# Autodesk Inventor assembly: Funnel Assembly
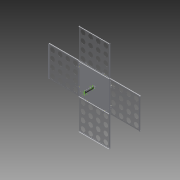
[picture p0: Inventor's stored thumbnail of the model, 180x180]
Saved by Autodesk Inventor 2014 (Build 180170000, 170)
## iProperties
Created: 2014-01-05
Part Number: Funnel Assembly
Document SubType Name: Assembly
Designer: Michael
Mass: 3587.59 g
Surface Area: 25589.4 cm^2
Volume: 1918.45 cm^3
Density: 1.87005 g/cm^3
Author: Michael
## Documents named in this file (5)
- C:\Users\Michael\Documents\Robotics\2014 Season\Funnel Catcher\Funnel Assembly.iam
- C:\Users\Michael\Documents\Robotics\2014 Season\Funnel Catcher\Funnel Plate Assembly.iam
- C:\Users\Michael\Documents\Robotics\2014 Season\Funnel Catcher\Flange for 3-4 in Piston.ipt
- C:\Users\Michael\Documents\Robotics\2014 Season\Funnel Catcher\9-16 in Pneumatic Cylinder (3 in Stroke).iam
- C:\Users\Michael\Documents\Robotics\2014 Season\Funnel Catcher\Back Funnel Piece.ipt
## Components (7 placed, 4 different names)
1. Funnel Plate Assembly:1 [sub-assembly] — Insert:3, Insert:4
2. Funnel Plate Assembly:3 [sub-assembly] — Insert:7, Insert:8
3. Funnel Plate Assembly:4 [sub-assembly] — Insert:5, Insert:6
4. Flange for 3-4 in Piston:1 — Insert:1, Insert:2, Insert:11, Insert:12
5. 9-16 in Pneumatic Cylinder (3 in Stroke):1 [sub-assembly] — Insert:1, Insert:2
6. Back Funnel Piece:1 — Insert:3, Insert:4, Insert:5, Insert:6, Insert:7, Insert:8, Insert:9, Insert:10, Insert:11, Insert:12
7. Funnel Plate Assembly:5 [sub-assembly] — Insert:9, Insert:10
## Relationships (12: Insert 12)
- Insert:1: Flange for 3-4 in Piston:1 ↔ 9-16 in Pneumatic Cylinder (3 in Stroke):1
- Insert:2: Flange for 3-4 in Piston:1 ↔ 9-16 in Pneumatic Cylinder (3 in Stroke):1
- Insert:3: Funnel Plate Assembly:1 ↔ Back Funnel Piece:1
- Insert:4: Funnel Plate Assembly:1 ↔ Back Funnel Piece:1
- Insert:5: Funnel Plate Assembly:4 ↔ Back Funnel Piece:1
- Insert:6: Funnel Plate Assembly:4 ↔ Back Funnel Piece:1
- Insert:7: Funnel Plate Assembly:3 ↔ Back Funnel Piece:1
- Insert:8: Funnel Plate Assembly:3 ↔ Back Funnel Piece:1
- Insert:9: Back Funnel Piece:1 ↔ Funnel Plate Assembly:5
- Insert:10: Back Funnel Piece:1 ↔ Funnel Plate Assembly:5
- Insert:11: Flange for 3-4 in Piston:1 ↔ Back Funnel Piece:1
- Insert:12: Flange for 3-4 in Piston:1 ↔ Back Funnel Piece:1
